# Autodesk Inventor assembly: EnsambleV2
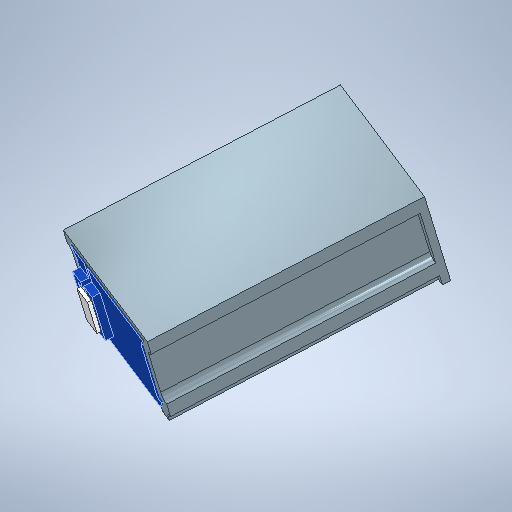
[picture p0: Inventor's stored thumbnail of the model, 512x512]
Saved by Autodesk Inventor 2025.1 (Build 291241020, 241B)
## iProperties
Created: 2024-09-01
Part Number: EnsambleV2
Document SubType Name: Assembly
Designer: andre
Author: andre
## Documents named in this file (6)
- C:\Users\andre\OneDrive_Personal\OneDrive\UCR\TCU\Diseño\EnsambleV2.iam
- C:\Users\andre\OneDrive_Personal\OneDrive\UCR\TCU\Diseño\CarcazaV2.ipt
- C:\Users\andre\OneDrive_Personal\OneDrive\UCR\TCU\Diseño\ESP32_DevBoard.ipt
- C:\Users\andre\OneDrive_Personal\OneDrive\UCR\TCU\Diseño\SecondCircuit.ipt
- C:\Users\andre\OneDrive_Personal\OneDrive\UCR\TCU\Diseño\SensorPin.ipt
- C:\Users\andre\OneDrive_Personal\OneDrive\UCR\TCU\Diseño\CarcasaSuperiorV2.ipt
## Components (5 placed, 5 different names)
1. CarcazaV2:1 — Mate:1, Mate:2, Mate:5, Mate:6, Mate:7, Mate:11, Mate:12, Mate:13
2. ESP32_DevBoard:1 — Mate:1, Mate:2, Mate:5
3. SecondCircuit:1 — Mate:6, Mate:7, Mate:8, Mate:9, Mate:10, Mate:11
4. SensorPin:1 — Mate:8, Mate:9, Mate:10
5. CarcasaSuperiorV2:1 — Mate:12, Mate:13
## Relationships (11: Mate 11)
- Mate:1: CarcazaV2:1 ↔ ESP32_DevBoard:1
- Mate:2: CarcazaV2:1 ↔ ESP32_DevBoard:1
- Mate:5 (0.25 mm): CarcazaV2:1 ↔ ESP32_DevBoard:1
- Mate:6: CarcazaV2:1 ↔ SecondCircuit:1
- Mate:7 (0.5 mm): CarcazaV2:1 ↔ SecondCircuit:1
- Mate:8: SecondCircuit:1 ↔ SensorPin:1
- Mate:9: SecondCircuit:1 ↔ SensorPin:1
- Mate:10: SecondCircuit:1 ↔ SensorPin:1
- Mate:11: CarcazaV2:1 ↔ SecondCircuit:1
- Mate:12: CarcazaV2:1 ↔ CarcasaSuperiorV2:1
- Mate:13: CarcazaV2:1 ↔ CarcasaSuperiorV2:1
